# Autodesk Inventor assembly: V
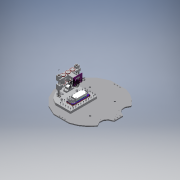
[picture p0: Inventor's stored thumbnail of the model, 180x180]
Saved by Autodesk Inventor 2017 (Build 210142000, 142)
## iProperties
Created: 2016-12-06
Part Number: V
Document SubType Name: Assembly
Designer: qupec
Mass: 1513.48 g
Surface Area: 2866.97 cm^2
Volume: 582.995 cm^3
Density: 2.59604 g/cm^3
Author: qupec
## Documents named in this file (36)
- C:\UMD\BPP\ROCKSAT X\STAR\CAD\Mechanical\Exploded Views\V.iam
- C:\UMD\BPP\ROCKSAT X\STAR\CAD\Mechanical\Full payload assembly\Subsystems\Slide Rods\Slide rod assembly.iam
- C:\UMD\BPP\ROCKSAT X\STAR\CAD\Mechanical\Full payload assembly\Subsystems\Test Tube Rack\Test tube rack.iam
- C:\UMD\BPP\ROCKSAT X\STAR\CAD\Mechanical\Full payload assembly\Subsystems\Electronics\Electronics Stack.iam
- C:\UMD\BPP\ROCKSAT X\STAR\CAD\Mechanical\Full payload assembly\Subsystems\Video Capture\Pi Cam and Cable assembly.iam
- C:\UMD\BPP\ROCKSAT X\STAR\CAD\Mechanical\Full payload assembly\Subsystems\Electronics\Ribbon Cable Connector-02.ipt
- C:\UMD\BPP\ROCKSAT X\STAR\CAD\Mechanical\Full payload assembly\Base Plate.ipt
- C:\UMD\BPP\ROCKSAT X\STAR\CAD\Mechanical\Full payload assembly\Subsystems\Electronics\External Sensor Board.ipt
- C:\UMD\BPP\ROCKSAT X\STAR\CAD\Mechanical\Full payload assembly\Subsystems\Video Capture\LED.ipt
- C:\UMD\BPP\ROCKSAT X\STAR\CAD\Mechanical\Full payload assembly\BRACKET.ipt
- C:\UMD\BPP\ROCKSAT X\STAR\CAD\Mechanical\Full payload assembly\Subsystems\Shaker\ShakerAssembly.iam
- C:\UMD\BPP\ROCKSAT X\STAR\CAD\Mechanical\Full payload assembly\Subsystems\Fasteners\Num4 Narrow Split Washer.ipt
- C:\UMD\BPP\ROCKSAT X\STAR\CAD\Mechanical\Full payload assembly\Subsystems\Fasteners\4-40 .5in Socket Screw.ipt
- C:\UMD\BPP\ROCKSAT X\STAR\CAD\Mechanical\Full payload assembly\Subsystems\Fasteners\4-40 .375in Countersunk Screw.ipt
- C:\UMD\BPP\ROCKSAT X\STAR\CAD\Mechanical\Full payload assembly\Subsystems\Fasteners\Num4 Flat Washer.ipt
- C:\UMD\BPP\ROCKSAT X\STAR\CAD\Mechanical\Full payload assembly\Subsystems\Fasteners\4-40 Flex Nut.ipt
- C:\UMD\BPP\ROCKSAT X\STAR\CAD\Mechanical\Full payload assembly\Subsystems\Fasteners\Num10 Belville Washer.ipt
- C:\UMD\BPP\ROCKSAT X\STAR\CAD\Mechanical\Full payload assembly\Subsystems\Fasteners\10-32 .375in Low Profile Socket Screw.ipt
- C:\UMD\BPP\ROCKSAT X\STAR\CAD\Mechanical\Full payload assembly\Subsystems\Fasteners\10-32 1.125in Countersunk Screw.ipt
- C:\UMD\BPP\ROCKSAT X\STAR\CAD\Mechanical\Full payload assembly\Subsystems\Fasteners\10-32 Flex Nut.ipt
- C:\UMD\BPP\ROCKSAT X\STAR\CAD\Mechanical\Full payload assembly\Subsystems\Fasteners\M2 Insulating Washer.ipt
- C:\UMD\BPP\ROCKSAT X\STAR\CAD\Mechanical\Full payload assembly\Subsystems\Fasteners\M2x.4mm Locknut.ipt
- C:\UMD\BPP\ROCKSAT X\STAR\CAD\Mechanical\Full payload assembly\Subsystems\Fasteners\M2x.4mm 12mm Socket Screw.ipt
- C:\UMD\BPP\ROCKSAT X\STAR\CAD\Mechanical\Full payload assembly\RSX Deck.ipt
- C:\UMD\BPP\ROCKSAT X\star\CAD\Mechanical\Subsystems\Full payload assembly mk 2\AIP\FEA\c3occb59c.fins
- C:\UMD\BPP\ROCKSAT X\star\CAD\Mechanical\Subsystems\Full payload assembly mk 2\AIP\FEA\c3occb5b4.fsat
- C:\UMD\BPP\ROCKSAT X\star\CAD\Mechanical\Subsystems\Full payload assembly mk 2\AIP\FEA\c3occb5b4.ftes
- C:\UMD\BPP\ROCKSAT X\star\CAD\Mechanical\Subsystems\Full payload assembly mk 2\AIP\FEA\c3occb5b4.fwiz
- C:\UMD\BPP\ROCKSAT X\star\CAD\Mechanical\Subsystems\Full payload assembly mk 2\AIP\FEA\c3occb5c0.fins
- C:\UMD\BPP\ROCKSAT X\star\CAD\Mechanical\Subsystems\Full payload assembly mk 2\AIP\FEA\c3occb5c0.fsat
- C:\UMD\BPP\ROCKSAT X\star\CAD\Mechanical\Subsystems\Full payload assembly mk 2\AIP\FEA\c3occb5c0.ftes
- C:\UMD\BPP\ROCKSAT X\star\CAD\Mechanical\Subsystems\Full payload assembly mk 2\AIP\FEA\c3occb5c0.fwiz
- C:\UMD\BPP\ROCKSAT X\star\CAD\Mechanical\Subsystems\Full payload assembly mk 2\AIP\FEA\c3occb60w.fmsh
- C:\UMD\BPP\ROCKSAT X\star\CAD\Mechanical\Subsystems\Full payload assembly mk 2\AIP\FEA\c3occb60x.fres
- C:\UMD\BPP\ROCKSAT X\star\CAD\Mechanical\Subsystems\Full payload assembly mk 2\AIP\FEA\c3occb6sg.fmsh
- C:\UMD\BPP\ROCKSAT X\star\CAD\Mechanical\Subsystems\Full payload assembly mk 2\AIP\FEA\c3occb6sh.fres
## Components (130 placed, 23 different names)
1. Slide rod assembly:1 [sub-assembly] — Mate:121, Mate:398, Mate:399
2. Test tube rack:1 [sub-assembly] — Mate:56, Flush:19, Flush:20, Flush:45, Mate:395, Mate:396, Mate:398, Mate:399, Mate:629, Mate:632, Mate:633, Mate:637, Mate:638
3. Pi Cam and Cable assembly:1 [sub-assembly] — Mate:56, Flush:19, Flush:20, Mate:299, Mate:300, Mate:302, Mate:303, Mate:593, Mate:594, Mate:595, Mate:596, Mate:597, Mate:598, Mate:599, Mate:600, Mate:606, Mate:625, Mate:626, Mate:627, Mate:628, Mate:630, Mate:631, Mate:636, Mate:654
4. Ribbon Cable Connector-02:1 — Mate:80, Flush:24, Flush:25
5. Electronics Stack:1 [sub-assembly] — Mate:80, Flush:24, Flush:25, Mate:397
6. Base Plate:1 — Mate:121, Mate:124, Flush:29, Flush:32, Flush:45, Mate:386, Mate:389, Mate:392, Mate:393, Mate:394, Mate:397, Mate:661, Mate:662, Mate:663, Mate:664, Mate:669, Mate:671, Mate:673
7. External Sensor Board:1 — Angle:1, Mate:303, Mate:305, Mate:306, Mate:609, Mate:610, Mate:611, Mate:612, Mate:613, Mate:614, Mate:615, Mate:616, Mate:646, Mate:647, Mate:648, Mate:649
8. LED:1 — Mate:299, Mate:301, Mate:302, Mate:305
9. LED:2 — Mate:300, Mate:301, Mate:306
10. BRACKET:1 — Mate:389, Mate:519, Mate:520, Mate:521, Mate:522, Mate:527, Mate:528, Mate:529, Mate:530
11. BRACKET:2 — Mate:386, Mate:523, Mate:524, Mate:525, Mate:526, Mate:531, Mate:532, Mate:533, Mate:534
12. ShakerAssembly:1 [sub-assembly] — Mate:392, Mate:393, Mate:394, Mate:395, Mate:396
13. Num4 Narrow Split Washer:1 — Mate:645
14. Num4 Narrow Split Washer:2
15. Num4 Narrow Split Washer:3
16. Num4 Narrow Split Washer:4
17. Num4 Narrow Split Washer:5
18. Num4 Narrow Split Washer:6
19. Num4 Narrow Split Washer:7
20. Num4 Narrow Split Washer:8
21. Num4 Narrow Split Washer:9
22. Num4 Narrow Split Washer:10
23. Num4 Narrow Split Washer:11
24. Num4 Narrow Split Washer:12
25. Num4 Narrow Split Washer:13
26. Num4 Narrow Split Washer:14
27. Num4 Narrow Split Washer:15
28. Num4 Narrow Split Washer:17
29. Num4 Narrow Split Washer:18
30. Num4 Narrow Split Washer:19
31. Num4 Narrow Split Washer:20
32. Num4 Narrow Split Washer:21
33. Num4 Narrow Split Washer:22
34. Num4 Narrow Split Washer:23
35. Num4 Narrow Split Washer:24
36. Num4 Narrow Split Washer:25
37. Num4 Narrow Split Washer:26
38. Num4 Narrow Split Washer:27
39. Num4 Narrow Split Washer:28
40. Num4 Narrow Split Washer:29
41. 4-40 .5in Socket Screw:1
42. 4-40 .5in Socket Screw:2
43. 4-40 .5in Socket Screw:3
44. 4-40 .5in Socket Screw:4
45. 4-40 .5in Socket Screw:5
46. 4-40 .5in Socket Screw:6
47. 4-40 .5in Socket Screw:7
48. 4-40 .5in Socket Screw:8
49. 4-40 .5in Socket Screw:9
50. 4-40 .5in Socket Screw:10
51. 4-40 .5in Socket Screw:11
52. 4-40 .5in Socket Screw:12
53. 4-40 .5in Socket Screw:13
54. 4-40 .5in Socket Screw:14
55. 4-40 .5in Socket Screw:15
56. 4-40 .5in Socket Screw:16
57. 4-40 .5in Socket Screw:17 — Mate:645
58. 4-40 .5in Socket Screw:18
59. 4-40 .5in Socket Screw:19
60. 4-40 .5in Socket Screw:20
61. 4-40 .5in Socket Screw:21
62. 4-40 .5in Socket Screw:22
63. 4-40 .5in Socket Screw:23
64. 4-40 .5in Socket Screw:24
65. 4-40 .5in Socket Screw:25
66. 4-40 .5in Socket Screw:26
67. 4-40 .5in Socket Screw:27
68. 4-40 .5in Socket Screw:28
69. 4-40 .375in Countersunk Screw:1 — Mate:520, Mate:521
70. 4-40 .375in Countersunk Screw:2 — Mate:519, Mate:522
71. 4-40 .375in Countersunk Screw:3 — Mate:523, Mate:526
72. 4-40 .375in Countersunk Screw:4 — Mate:524, Mate:525
73. 4-40 .375in Countersunk Screw:5 — Mate:531, Mate:534, Mate:537, Mate:546
74. 4-40 .375in Countersunk Screw:6 — Mate:528, Mate:529, Mate:541, Mate:550
75. 4-40 .375in Countersunk Screw:7 — Mate:532, Mate:533, Mate:535, Mate:543
76. 4-40 .375in Countersunk Screw:8 — Mate:527, Mate:530, Mate:539, Mate:548
77. Num4 Flat Washer:1 — Mate:539, Mate:660
78. Num4 Flat Washer:2 — Mate:537, Mate:658
79. Num4 Flat Washer:3 — Mate:535, Mate:659
80. Num4 Flat Washer:4 — Mate:541, Mate:657
81. 4-40 Flex Nut:1 — Mate:550, Mate:657
82. 4-40 Flex Nut:2 — Mate:546, Mate:658
83. 4-40 Flex Nut:3 — Mate:548, Mate:660
84. 4-40 Flex Nut:4 — Mate:543, Mate:659
85. Num4 Narrow Split Washer:30
86. Num10 Belville Washer:1 — Mate:574
87. Num10 Belville Washer:3 — Mate:573
88. Num10 Belville Washer:4 — Mate:572
89. 10-32 .375in Low Profile Socket Screw:1 — Mate:574
90. 10-32 .375in Low Profile Socket Screw:2 — Mate:573, Mate:670, Mate:671
91. 10-32 .375in Low Profile Socket Screw:3 — Mate:572
92. 10-32 1.125in Countersunk Screw:1 — Mate:585
93. 10-32 1.125in Countersunk Screw:2 — Mate:587, Mate:672, Mate:673, Mate:674
94. 10-32 1.125in Countersunk Screw:3 — Mate:586
95. 10-32 1.125in Countersunk Screw:4 — Mate:588
96. 10-32 Flex Nut:1 — Mate:586, Mate:661
97. 10-32 Flex Nut:2 — Mate:587, Mate:662, Mate:674
98. 10-32 Flex Nut:3 — Mate:588, Mate:664
99. 10-32 Flex Nut:4 — Mate:585, Mate:663
100. M2 Insulating Washer:1 — Mate:593, Mate:594, Mate:603, Mate:665
101. M2 Insulating Washer:2 — Mate:599, Mate:600, Mate:608, Mate:668
102. M2 Insulating Washer:3 — Mate:597, Mate:598, Mate:667
103. M2 Insulating Washer:4 — Mate:595, Mate:596, Mate:602, Mate:666
104. M2x.4mm Locknut:1 — Mate:602, Mate:666
105. M2x.4mm Locknut:2 — Mate:603, Mate:665
106. M2x.4mm Locknut:3 — Mate:608, Mate:668
107. M2x.4mm Locknut:4 — Mate:606, Mate:667
108. M2x.4mm 12mm Socket Screw:1 — Mate:610, Mate:619, Mate:623, Mate:652
109. M2x.4mm 12mm Socket Screw:2 — Mate:609, Mate:618, Mate:621, Mate:653
110. M2x.4mm 12mm Socket Screw:3 — Mate:611, Mate:617, Mate:622, Mate:650
111. M2x.4mm 12mm Socket Screw:4 — Mate:612, Mate:620, Mate:624, Mate:651
112. M2 Insulating Washer:5 — Mate:616, Mate:617
113. M2 Insulating Washer:6 — Mate:614, Mate:619
114. M2 Insulating Washer:7 — Mate:613, Mate:620, Mate:624
115. M2 Insulating Washer:8 — Mate:615, Mate:618, Mate:621, Mate:622, Mate:623
116. Num4 Flat Washer:5 — Mate:625, Mate:630, Mate:634, Mate:635
117. Num4 Flat Washer:6 — Mate:627, Mate:629
118. Num4 Flat Washer:7 — Mate:626, Mate:628
119. 4-40 .5in Socket Screw:29 — Mate:631, Mate:636, Mate:639, Mate:644
120. 4-40 .5in Socket Screw:30 — Mate:632, Mate:634, Mate:640, Mate:643
121. 4-40 .5in Socket Screw:31 — Mate:633, Mate:635
122. Num4 Flat Washer:8 — Mate:637, Mate:640, Mate:656
123. Num4 Flat Washer:9 — Mate:638, Mate:639, Mate:655
124. 4-40 Flex Nut:5 — Mate:643, Mate:656
125. 4-40 Flex Nut:6 — Mate:644, Mate:655
126. M2 Insulating Washer:9 — Mate:647, Mate:650, Mate:654
127. M2 Insulating Washer:10 — Mate:646, Mate:651
128. M2 Insulating Washer:11 — Mate:649, Mate:653
129. M2 Insulating Washer:12 — Mate:648, Mate:652
130. RSX Deck:1 — Mate:669, Mate:670, Mate:672
## Relationships (180: Mate 172, Flush 7, Angle 1)
- Mate:56: Test tube rack:1 ↔ Pi Cam and Cable assembly:1
- Flush:19: Test tube rack:1 ↔ Pi Cam and Cable assembly:1
- Flush:20: Test tube rack:1 ↔ Pi Cam and Cable assembly:1
- Mate:80: Ribbon Cable Connector-02:1 ↔ Electronics Stack:1
- Flush:24 (-7 mm): Ribbon Cable Connector-02:1 ↔ Electronics Stack:1
- Flush:25: Ribbon Cable Connector-02:1 ↔ Electronics Stack:1
- Mate:121: Slide rod assembly:1 ↔ Base Plate:1
- Mate:124: Base Plate:1
- Flush:29: Base Plate:1
- Flush:32: Base Plate:1
- Angle:1 (0 deg): External Sensor Board:1
- Mate:299: Pi Cam and Cable assembly:1 ↔ LED:1
- Mate:300: Pi Cam and Cable assembly:1 ↔ LED:2
- Mate:301: LED:1 ↔ LED:2
- Mate:302: Pi Cam and Cable assembly:1 ↔ LED:1
- Mate:303: Pi Cam and Cable assembly:1 ↔ External Sensor Board:1
- Mate:305: External Sensor Board:1 ↔ LED:1
- Mate:306: External Sensor Board:1 ↔ LED:2
- Flush:45: Test tube rack:1 ↔ Base Plate:1
- Mate:386: Base Plate:1 ↔ BRACKET:2
- Mate:389: Base Plate:1 ↔ BRACKET:1
- Mate:392: Base Plate:1 ↔ ShakerAssembly:1
- Mate:393: Base Plate:1 ↔ ShakerAssembly:1
- Mate:394: Base Plate:1 ↔ ShakerAssembly:1
- Mate:395: Test tube rack:1 ↔ ShakerAssembly:1
- Mate:396: Test tube rack:1 ↔ ShakerAssembly:1
- Mate:397: Electronics Stack:1 ↔ Base Plate:1
- Mate:398: Slide rod assembly:1 ↔ Test tube rack:1
- Mate:399: Slide rod assembly:1 ↔ Test tube rack:1
- [Mate]: Num4 Narrow Split Washer:29 ↔ 4-40 .5in Socket Screw:13
- [Mate]: Num4 Narrow Split Washer:4 ↔ 4-40 .5in Socket Screw:5
- [Mate]: Num4 Narrow Split Washer:20 ↔ 4-40 .5in Socket Screw:4
- [Mate]: Num4 Narrow Split Washer:9 ↔ 4-40 .5in Socket Screw:26
- [Mate]: Num4 Narrow Split Washer:14 ↔ 4-40 .5in Socket Screw:1
- [Mate]: Num4 Narrow Split Washer:21 ↔ 4-40 .5in Socket Screw:11
- [Mate]: Num4 Narrow Split Washer:13 ↔ 4-40 .5in Socket Screw:2
- [Mate]: Num4 Narrow Split Washer:22 ↔ 4-40 .5in Socket Screw:23
- [Mate]: Num4 Narrow Split Washer:18 ↔ 4-40 .5in Socket Screw:22
- [Mate]: Num4 Narrow Split Washer:15 ↔ 4-40 .5in Socket Screw:28
- [Mate]: Num4 Narrow Split Washer:24 ↔ 4-40 .5in Socket Screw:16
- [Mate]: Num4 Narrow Split Washer:8 ↔ 4-40 .5in Socket Screw:14
- [Mate]: Num4 Narrow Split Washer:25 ↔ 4-40 .5in Socket Screw:15
- [Mate]: Num4 Narrow Split Washer:6 ↔ 4-40 .5in Socket Screw:24
- [Mate]: Num4 Narrow Split Washer:11 ↔ 4-40 .5in Socket Screw:9
- [Mate]: Num4 Narrow Split Washer:27 ↔ 4-40 .5in Socket Screw:21
- [Mate]: Num4 Narrow Split Washer:12 ↔ 4-40 .5in Socket Screw:18
- [Mate]: Num4 Narrow Split Washer:28 ↔ 4-40 .5in Socket Screw:19
- [Mate]: Num4 Narrow Split Washer:26 ↔ 4-40 .5in Socket Screw:20
- [Mate]: Num4 Narrow Split Washer:3 ↔ 4-40 .5in Socket Screw:25
- [Mate]: Num4 Narrow Split Washer:10 ↔ 4-40 .5in Socket Screw:8
- [Mate]: Num4 Narrow Split Washer:5 ↔ 4-40 .5in Socket Screw:10
- [Mate]: Num4 Narrow Split Washer:7 ↔ 4-40 .5in Socket Screw:7
- [Mate]: Num4 Narrow Split Washer:17 ↔ 4-40 .5in Socket Screw:3
- [Mate]: Num4 Narrow Split Washer:2 ↔ 4-40 .5in Socket Screw:12
- [Mate]: Num4 Narrow Split Washer:19 ↔ 4-40 .5in Socket Screw:6
- [Mate]: Num4 Narrow Split Washer:1 ↔ 4-40 .5in Socket Screw:17
- [Mate]: Num4 Narrow Split Washer:14 ↔ 4-40 .5in Socket Screw:1
- [Mate]: Num4 Narrow Split Washer:9 ↔ 4-40 .5in Socket Screw:26
- [Mate]: Num4 Narrow Split Washer:23 ↔ 4-40 .5in Socket Screw:27
- [Mate]: Num4 Narrow Split Washer:20 ↔ 4-40 .5in Socket Screw:4
- [Mate]: Num4 Narrow Split Washer:4 ↔ 4-40 .5in Socket Screw:5
- [Mate]: Num4 Narrow Split Washer:29 ↔ 4-40 .5in Socket Screw:13
- [Mate]: Num4 Narrow Split Washer:11 ↔ 4-40 .5in Socket Screw:9
- [Mate]: Num4 Narrow Split Washer:27 ↔ 4-40 .5in Socket Screw:21
- [Mate]: Num4 Narrow Split Washer:12 ↔ 4-40 .5in Socket Screw:18
- [Mate]: Num4 Narrow Split Washer:28 ↔ 4-40 .5in Socket Screw:19
- [Mate]: Num4 Narrow Split Washer:26 ↔ 4-40 .5in Socket Screw:20
- [Mate]: Num4 Narrow Split Washer:3 ↔ 4-40 .5in Socket Screw:25
- [Mate]: Num4 Narrow Split Washer:7 ↔ 4-40 .5in Socket Screw:7
- [Mate]: Num4 Narrow Split Washer:17 ↔ 4-40 .5in Socket Screw:3
- [Mate]: Num4 Narrow Split Washer:2 ↔ 4-40 .5in Socket Screw:12
- [Mate]: Num4 Narrow Split Washer:19 ↔ 4-40 .5in Socket Screw:6
- [Mate]: Num4 Narrow Split Washer:29 ↔ 4-40 .5in Socket Screw:13
- Mate:519: BRACKET:1 ↔ 4-40 .375in Countersunk Screw:2
- Mate:520: BRACKET:1 ↔ 4-40 .375in Countersunk Screw:1
- Mate:521: BRACKET:1 ↔ 4-40 .375in Countersunk Screw:1
- Mate:522: BRACKET:1 ↔ 4-40 .375in Countersunk Screw:2
- Mate:523: BRACKET:2 ↔ 4-40 .375in Countersunk Screw:3
- Mate:524: BRACKET:2 ↔ 4-40 .375in Countersunk Screw:4
- Mate:525: BRACKET:2 ↔ 4-40 .375in Countersunk Screw:4
- Mate:526: BRACKET:2 ↔ 4-40 .375in Countersunk Screw:3
- Mate:527: BRACKET:1 ↔ 4-40 .375in Countersunk Screw:8
- Mate:528: BRACKET:1 ↔ 4-40 .375in Countersunk Screw:6
- Mate:529: BRACKET:1 ↔ 4-40 .375in Countersunk Screw:6
- Mate:530: BRACKET:1 ↔ 4-40 .375in Countersunk Screw:8
- Mate:531: BRACKET:2 ↔ 4-40 .375in Countersunk Screw:5
- Mate:532: BRACKET:2 ↔ 4-40 .375in Countersunk Screw:7
- Mate:533: BRACKET:2 ↔ 4-40 .375in Countersunk Screw:7
- Mate:534: BRACKET:2 ↔ 4-40 .375in Countersunk Screw:5
- Mate:535: 4-40 .375in Countersunk Screw:7 ↔ Num4 Flat Washer:3
- Mate:537: 4-40 .375in Countersunk Screw:5 ↔ Num4 Flat Washer:2
- Mate:539: 4-40 .375in Countersunk Screw:8 ↔ Num4 Flat Washer:1
- Mate:541: 4-40 .375in Countersunk Screw:6 ↔ Num4 Flat Washer:4
- Mate:543: 4-40 .375in Countersunk Screw:7 ↔ 4-40 Flex Nut:4
- Mate:546: 4-40 .375in Countersunk Screw:5 ↔ 4-40 Flex Nut:2
- Mate:548: 4-40 .375in Countersunk Screw:8 ↔ 4-40 Flex Nut:3
- Mate:550: 4-40 .375in Countersunk Screw:6 ↔ 4-40 Flex Nut:1
- Mate:572: Num10 Belville Washer:4 ↔ 10-32 .375in Low Profile Socket Screw:3
- Mate:573: Num10 Belville Washer:3 ↔ 10-32 .375in Low Profile Socket Screw:2
- Mate:574: Num10 Belville Washer:1 ↔ 10-32 .375in Low Profile Socket Screw:1
- Mate:585: 10-32 1.125in Countersunk Screw:1 ↔ 10-32 Flex Nut:4
- Mate:586: 10-32 1.125in Countersunk Screw:3 ↔ 10-32 Flex Nut:1
- Mate:587: 10-32 1.125in Countersunk Screw:2 ↔ 10-32 Flex Nut:2
- Mate:588: 10-32 1.125in Countersunk Screw:4 ↔ 10-32 Flex Nut:3
- Mate:593: Pi Cam and Cable assembly:1 ↔ M2 Insulating Washer:1
- Mate:594: Pi Cam and Cable assembly:1 ↔ M2 Insulating Washer:1
- Mate:595: Pi Cam and Cable assembly:1 ↔ M2 Insulating Washer:4
- Mate:596: Pi Cam and Cable assembly:1 ↔ M2 Insulating Washer:4
- Mate:597: Pi Cam and Cable assembly:1 ↔ M2 Insulating Washer:3
- Mate:598: Pi Cam and Cable assembly:1 ↔ M2 Insulating Washer:3
- Mate:599: Pi Cam and Cable assembly:1 ↔ M2 Insulating Washer:2
- Mate:600: Pi Cam and Cable assembly:1 ↔ M2 Insulating Washer:2
- Mate:602: M2 Insulating Washer:4 ↔ M2x.4mm Locknut:1
- Mate:603: M2 Insulating Washer:1 ↔ M2x.4mm Locknut:2
- Mate:606: Pi Cam and Cable assembly:1 ↔ M2x.4mm Locknut:4
- Mate:608: M2 Insulating Washer:2 ↔ M2x.4mm Locknut:3
- Mate:609: External Sensor Board:1 ↔ M2x.4mm 12mm Socket Screw:2
- Mate:610: External Sensor Board:1 ↔ M2x.4mm 12mm Socket Screw:1
- Mate:611: External Sensor Board:1 ↔ M2x.4mm 12mm Socket Screw:3
- Mate:612: External Sensor Board:1 ↔ M2x.4mm 12mm Socket Screw:4
- Mate:613: External Sensor Board:1 ↔ M2 Insulating Washer:7
- Mate:614: External Sensor Board:1 ↔ M2 Insulating Washer:6
- Mate:615: External Sensor Board:1 ↔ M2 Insulating Washer:8
- Mate:616: External Sensor Board:1 ↔ M2 Insulating Washer:5
- Mate:617: M2x.4mm 12mm Socket Screw:3 ↔ M2 Insulating Washer:5
- Mate:618: M2x.4mm 12mm Socket Screw:2 ↔ M2 Insulating Washer:8
- Mate:619: M2x.4mm 12mm Socket Screw:1 ↔ M2 Insulating Washer:6
- Mate:620: M2x.4mm 12mm Socket Screw:4 ↔ M2 Insulating Washer:7
- Mate:621: M2x.4mm 12mm Socket Screw:2 ↔ M2 Insulating Washer:8
- Mate:622: M2x.4mm 12mm Socket Screw:3 ↔ M2 Insulating Washer:8
- Mate:623: M2x.4mm 12mm Socket Screw:1 ↔ M2 Insulating Washer:8
- Mate:624: M2x.4mm 12mm Socket Screw:4 ↔ M2 Insulating Washer:7
- Mate:625: Pi Cam and Cable assembly:1 ↔ Num4 Flat Washer:5
- Mate:626: Pi Cam and Cable assembly:1 ↔ Num4 Flat Washer:7
- Mate:627: Pi Cam and Cable assembly:1 ↔ Num4 Flat Washer:6
- Mate:628: Pi Cam and Cable assembly:1 ↔ Num4 Flat Washer:7
- Mate:629: Test tube rack:1 ↔ Num4 Flat Washer:6
- Mate:630: Pi Cam and Cable assembly:1 ↔ Num4 Flat Washer:5
- Mate:631: Pi Cam and Cable assembly:1 ↔ 4-40 .5in Socket Screw:29
- Mate:632: Test tube rack:1 ↔ 4-40 .5in Socket Screw:30
- Mate:633: Test tube rack:1 ↔ 4-40 .5in Socket Screw:31
- Mate:634: Num4 Flat Washer:5 ↔ 4-40 .5in Socket Screw:30
- Mate:635: Num4 Flat Washer:5 ↔ 4-40 .5in Socket Screw:31
- Mate:636: Pi Cam and Cable assembly:1 ↔ 4-40 .5in Socket Screw:29
- Mate:637: Test tube rack:1 ↔ Num4 Flat Washer:8
- Mate:638: Test tube rack:1 ↔ Num4 Flat Washer:9
- Mate:639: 4-40 .5in Socket Screw:29 ↔ Num4 Flat Washer:9
- Mate:640: 4-40 .5in Socket Screw:30 ↔ Num4 Flat Washer:8
- Mate:643: 4-40 .5in Socket Screw:30 ↔ 4-40 Flex Nut:5
- Mate:644: 4-40 .5in Socket Screw:29 ↔ 4-40 Flex Nut:6
- Mate:645: Num4 Narrow Split Washer:1 ↔ 4-40 .5in Socket Screw:17
- Mate:646: External Sensor Board:1 ↔ M2 Insulating Washer:10
- Mate:647: External Sensor Board:1 ↔ M2 Insulating Washer:9
- Mate:648: External Sensor Board:1 ↔ M2 Insulating Washer:12
- Mate:649: External Sensor Board:1 ↔ M2 Insulating Washer:11
- Mate:650: M2x.4mm 12mm Socket Screw:3 ↔ M2 Insulating Washer:9
- Mate:651: M2x.4mm 12mm Socket Screw:4 ↔ M2 Insulating Washer:10
- Mate:652: M2x.4mm 12mm Socket Screw:1 ↔ M2 Insulating Washer:12
- Mate:653: M2x.4mm 12mm Socket Screw:2 ↔ M2 Insulating Washer:11
- Mate:654: Pi Cam and Cable assembly:1 ↔ M2 Insulating Washer:9
- Mate:655: Num4 Flat Washer:9 ↔ 4-40 Flex Nut:6
- Mate:656: Num4 Flat Washer:8 ↔ 4-40 Flex Nut:5
- Mate:657: Num4 Flat Washer:4 ↔ 4-40 Flex Nut:1
- Mate:658: Num4 Flat Washer:2 ↔ 4-40 Flex Nut:2
- Mate:659: Num4 Flat Washer:3 ↔ 4-40 Flex Nut:4
- Mate:660: Num4 Flat Washer:1 ↔ 4-40 Flex Nut:3
- Mate:661: Base Plate:1 ↔ 10-32 Flex Nut:1
- Mate:662: Base Plate:1 ↔ 10-32 Flex Nut:2
- Mate:663: Base Plate:1 ↔ 10-32 Flex Nut:4
- Mate:664: Base Plate:1 ↔ 10-32 Flex Nut:3
- Mate:665: M2 Insulating Washer:1 ↔ M2x.4mm Locknut:2
- Mate:666: M2 Insulating Washer:4 ↔ M2x.4mm Locknut:1
- Mate:667: M2 Insulating Washer:3 ↔ M2x.4mm Locknut:4
- Mate:668: M2 Insulating Washer:2 ↔ M2x.4mm Locknut:3
- Mate:669: Base Plate:1 ↔ RSX Deck:1
- Mate:670: 10-32 .375in Low Profile Socket Screw:2 ↔ RSX Deck:1
- Mate:671: Base Plate:1 ↔ 10-32 .375in Low Profile Socket Screw:2
- Mate:672: 10-32 1.125in Countersunk Screw:2 ↔ RSX Deck:1
- Mate:673: Base Plate:1 ↔ 10-32 1.125in Countersunk Screw:2
- Mate:674: 10-32 1.125in Countersunk Screw:2 ↔ 10-32 Flex Nut:2
## Named parameters: sa_3 = 0, sa_4 = 29260.8, sa_5 = 0, sa_6 = 6894.76
note: some values were not read from the file. Shown as the stored number, unit unknown: "sa_3", "sa_4", "sa_5", "sa_6".
